# Autodesk Inventor assembly: 3030_L-Bracket_asm.ipt
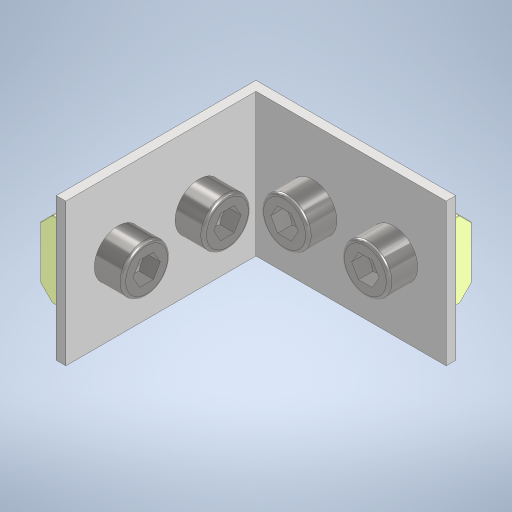
[picture p0: Inventor's stored thumbnail of the model, 512x512]
Saved by Autodesk Inventor 2024 (Build 280153000, 153)
## iProperties
Created: 2025-12-17
Part Number: 3030_L-Bracket_asm.ipt
Document SubType Name: Assembly
Designer: schar
Author: schar
## Documents named in this file (4)
- C:\Users\schar\Desktop\projectBlueprint\AMSTS\hardware\3030_L-Bracket_asm.ipt.iam
- C:\Users\schar\Desktop\projectBlueprint\AMSTS\hardware\3030_L-Bracket.ipt
- C:\Users\schar\Desktop\projectBlueprint\AMSTS\hardware\3030_tnut_m6_MIR.ipt
- C:\Users\schar\Documents\Inventor\Content Center Files\R2024\en-US\ISO 4762(1)\DIN EN ISO 4762 - M6 x 10.ipt
## Components (9 placed, 3 different names)
1. 3030_L-Bracket:1 — Rotational:1, Rotational:2, Rotational:3, Rotational:4, Mate:5, Mate:6, Mate:7, Mate:8
2. 3030_tnut_m6_MIR:1 — Rotational:1, Mate:1
3. 3030_tnut_m6_MIR:2 — Rotational:2, Mate:2
4. 3030_tnut_m6_MIR:3 — Rotational:3, Mate:3
5. 3030_tnut_m6_MIR:4 — Rotational:4, Mate:4
6. DIN EN ISO 4762 M6 x 10:1 — Mate:1, Mate:8
7. DIN EN ISO 4762 M6 x 10:2 — Mate:2, Mate:7
8. DIN EN ISO 4762 M6 x 10:3 — Mate:3, Mate:6
9. DIN EN ISO 4762 M6 x 10:4 — Mate:4, Mate:5
## Relationships (12: Mate 8, RevoluteJoint 4)
- Rotational:1 [RevoluteJoint] (-0.357 mm): 3030_L-Bracket:1 ↔ 3030_tnut_m6_MIR:1
- Rotational:2 [RevoluteJoint] (-0.357 mm): 3030_L-Bracket:1 ↔ 3030_tnut_m6_MIR:2
- Rotational:3 [RevoluteJoint] (-0.357 mm): 3030_L-Bracket:1 ↔ 3030_tnut_m6_MIR:3
- Rotational:4 [RevoluteJoint] (-0.357 mm): 3030_L-Bracket:1 ↔ 3030_tnut_m6_MIR:4
- Mate:1: 3030_tnut_m6_MIR:1 ↔ DIN EN ISO 4762 M6 x 10:1
- Mate:2: 3030_tnut_m6_MIR:2 ↔ DIN EN ISO 4762 M6 x 10:2
- Mate:3: 3030_tnut_m6_MIR:3 ↔ DIN EN ISO 4762 M6 x 10:3
- Mate:4: 3030_tnut_m6_MIR:4 ↔ DIN EN ISO 4762 M6 x 10:4
- Mate:5: 3030_L-Bracket:1 ↔ DIN EN ISO 4762 M6 x 10:4
- Mate:6: 3030_L-Bracket:1 ↔ DIN EN ISO 4762 M6 x 10:3
- Mate:7: 3030_L-Bracket:1 ↔ DIN EN ISO 4762 M6 x 10:2
- Mate:8: 3030_L-Bracket:1 ↔ DIN EN ISO 4762 M6 x 10:1
